# Autodesk Inventor assembly: DriveBase2020
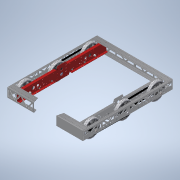
[picture p0: Inventor's stored thumbnail of the model, 180x180]
Saved by Autodesk Inventor 2020 (Build 240168000, 168)
## iProperties
Created: 2017-12-15
Part Number: DriveBase2020
Document SubType Name: Assembly
Designer: Autodesk Inc.
Catalog Web Link: http://www.andymark.com/AM14U3-p/am-14u3.htm
Vendor: Andy Mark Inc.
Category: Drive Base
Company: Autodesk Inc.
Author: Autodesk Inc.
Keywords: Drive Base Long
## Documents named in this file (5)
- C:\Users\srini\Documents\FRC\2020\DriveBase2020.iam
- C:\Users\srini\Documents\FRC\2020\2018_KOP\Inventor\FRC 2018 Drive Base Inventor\FIRST 2018 Drive Base\Parts\AM14U3 Long Half.iam
- C:\Users\srini\Documents\FRC\2020\2018_KOP\Inventor\FRC 2018 Drive Base Inventor\FIRST 2018 Drive Base\Parts\AM14U3 End Sheet Square.ipt
- C:\Users\srini\Documents\FRC\2020\2018_KOP\Inventor\FRC 2018 Drive Base Inventor\FIRST 2018 Drive Base\Parts\AM14U3 End Sheet PowerCell.ipt
- C:\Users\srini\Documents\FRC\2020\2018_KOP\Inventor\FRC 2018 Drive Base Inventor\FIRST 2018 Drive Base\Parts\AM14U3 End Sheet PowerCell_MIR.ipt
## Components (5 placed, 5 different names)
1. AM14U3 Long Half_1 [sub-assembly] — Mate:1, Flush:1, Insert:1, Insert:2, Insert:7, Insert:8
2. AM14U3 Long Half:2 [sub-assembly] — Flush:1, Insert:3, Insert:4, Insert:5, Insert:6
3. AM14U3 End Sheet Square:2 — Insert:1, Insert:2, Insert:5, Insert:6
4. AM14U3 End Sheet PowerCell:1 — Insert:3, Insert:4
5. AM14U3 End Sheet PowerCell_MIR:1 — Insert:7, Insert:8
## Relationships (10: Insert 8, Mate 1, Flush 1)
- Mate:1: AM14U3 Long Half_1
- Flush:1: AM14U3 Long Half_1 ↔ AM14U3 Long Half:2
- Insert:1: AM14U3 Long Half_1 ↔ AM14U3 End Sheet Square:2
- Insert:2: AM14U3 Long Half_1 ↔ AM14U3 End Sheet Square:2
- Insert:3: AM14U3 Long Half:2 ↔ AM14U3 End Sheet PowerCell:1
- Insert:4: AM14U3 Long Half:2 ↔ AM14U3 End Sheet PowerCell:1
- Insert:5: AM14U3 Long Half:2 ↔ AM14U3 End Sheet Square:2
- Insert:6: AM14U3 Long Half:2 ↔ AM14U3 End Sheet Square:2
- Insert:7: AM14U3 Long Half_1 ↔ AM14U3 End Sheet PowerCell_MIR:1
- Insert:8: AM14U3 Long Half_1 ↔ AM14U3 End Sheet PowerCell_MIR:1
